# Autodesk Inventor assembly: Turntable-ArmConnection
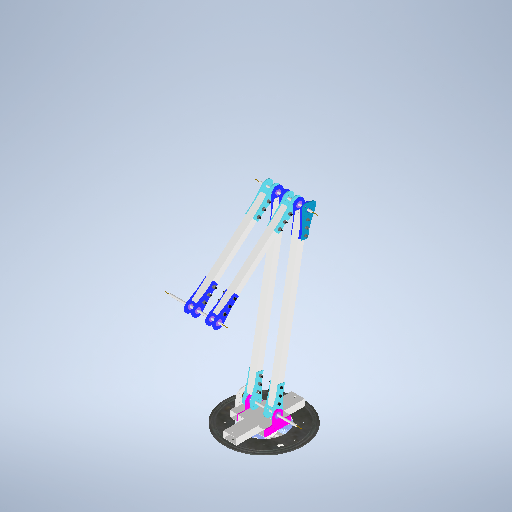
[picture p0: Inventor's stored thumbnail of the model, 512x512]
Saved by Autodesk Inventor 2025.1 (Build 291241000, 241)
## iProperties
Created: 2024-01-10
Part Number: Turntable-ArmConnection
Document SubType Name: Assembly
Designer: megan
Author: megan
## Documents named in this file (18)
- C:\Users\ejned\OneDrive - The Pennsylvania State University\BehrendURCMechanical\CAD\Apparatus\Arm Base\Arm.iam
- C:\Users\ejned\OneDrive - The Pennsylvania State University\BehrendURCMechanical\CAD\Apparatus\Arm Base\1544T3_Lubricated Turntable.ipt
- C:\Users\ejned\OneDrive - The Pennsylvania State University\BehrendURCMechanical\CAD\Apparatus\Arm Base\2inTubeBase.ipt
- C:\Users\ejned\OneDrive - The Pennsylvania State University\BehrendURCMechanical\CAD\Apparatus\Arm Base\1inTubeBase.ipt
- C:\Users\ejned\OneDrive - The Pennsylvania State University\BehrendURCMechanical\CAD\Apparatus\Arm Base\ArmPlateBase.ipt
- C:\Users\ejned\OneDrive - The Pennsylvania State University\BehrendURCMechanical\CAD\Apparatus\Arm Base\JointShaft.ipt
- C:\Users\ejned\OneDrive - The Pennsylvania State University\BehrendURCMechanical\CAD\Chassis V3\Arm Plate2.ipt
- C:\Users\ejned\OneDrive - The Pennsylvania State University\BehrendURCMechanical\CAD\Chassis V3\24in long 1in square tube.ipt
- C:\Users\ejned\OneDrive - The Pennsylvania State University\BehrendURCMechanical\CAD\Apparatus\Arm Base\8mmBearing.ipt
- C:\Users\ejned\OneDrive - The Pennsylvania State University\BehrendURCMechanical\CAD\Chassis V3\Arm Plate.ipt
- C:\Users\ejned\OneDrive - The Pennsylvania State University\BehrendURCMechanical\CAD\Chassis V3\14in long 1in square tube.ipt
- C:\Users\ejned\OneDrive - The Pennsylvania State University\BehrendURCMechanical\CAD\Chassis V3\Bolt Nut Washer assem.iam
- C:\Users\ejned\OneDrive - The Pennsylvania State University\BehrendURCMechanical\CAD\Apparatus\Arm Base\AP-0-02-baseAllTry2.iam
- C:\Users\ejned\OneDrive - The Pennsylvania State University\BehrendURCMechanical\CAD\Chassis V3\90107A011_316 Stainless Steel Washer.ipt
- C:\Users\ejned\OneDrive - The Pennsylvania State University\BehrendURCMechanical\CAD\Chassis V3\Arm Plate4.ipt
- C:\Users\ejned\OneDrive - The Pennsylvania State University\BehrendURCMechanical\CAD\Apparatus\91290A198_Alloy Steel Socket Head Screw.ipt
- C:\Users\ejned\OneDrive - The Pennsylvania State University\BehrendURCMechanical\CAD\Chassis V3\91831A011_18-8 Stainless Steel Nylon-Insert Locknut.ipt
- C:\Users\ejned\OneDrive - The Pennsylvania State University\BehrendURCMechanical\CAD\Apparatus\Arm Base\ArmPlateBase V2.ipt
## Components (76 placed, 15 different names)
1. 1544T3_Lubricated Turntable:1 — Mate:3, Mate:197, Mate:198, Mate:199, Mate:201
2. AP-0-02-baseAllTry2:1 [sub-assembly] — Mate:199
3. ArmPlateBase V2:1 — Rotational:1
4. ArmPlateBase:1 — Mate:57, Mate:58, Mate:59, Mate:60, Mate:63, Mate:65, Mate:271, Mate:272, Mate:273
5. ArmPlateBase:2 — Mate:61, Mate:62, Flush:5, Mate:66
6. arm plate:1 — Mate:22, Mate:73, Mate:74, Mate:142, Mate:143, Mate:150, Mate:151, Mate:152, Mate:153
7. arm plate:3 — Mate:80, Mate:81, Mate:204, Mate:207, Mate:236, Mate:237
8. arm plate:4 — Mate:49, Mate:50, Mate:51, Mate:213, Mate:262, Mate:264, Mate:266
9. arm plate:5 — Mate:67, Mate:68, Mate:69, Mate:77, Mate:78, Mate:154, Mate:155, Mate:156, Mate:157, Mate:168, Mate:169, Mate:284
10. arm plate:6 — Mate:70, Mate:71, Mate:72, Mate:79, Mate:82, Mate:283
11. arm plate:7 — Mate:84, Mate:86
12. arm plate:8 — Mate:83, Mate:85
13. arm plate:10 — Mate:93, Mate:104, Mate:105, Mate:170, Mate:171, Mate:172, Mate:173, Mate:174, Mate:175, Mate:283
14. arm plate:11 — Mate:95, Mate:101, Flush:7, Mate:159, Mate:284
15. arm plate:12 — Mate:97, Mate:103, Mate:160
16. arm plate:13 — Mate:106, Mate:107, Mate:111, Mate:115, Mate:117, Mate:124, Mate:188, Mate:189, Mate:190, Mate:191, Mate:192, Mate:193
17. arm plate:14 — Mate:108, Mate:109, Mate:114, Mate:122
18. arm plate:15 — Mate:110, Mate:111, Mate:116, Mate:120
19. arm plate:16 — Mate:112, Mate:113, Flush:9, Mate:118, Mate:182, Mate:183, Mate:184, Mate:185, Mate:186, Mate:187
20. arm plate:18 — Mate:226, Mate:227, Mate:228, Mate:229, Mate:230, Mate:231, Mate:232, Mate:233, Mate:234
21. arm plate:19 — Mate:235, Mate:236, Mate:237, Mate:243, Mate:244, Mate:245, Mate:247, Mate:248, Mate:251, Mate:252, Mate:253, Mate:255, Mate:256, Mate:258, Mate:260, Flush:13
22. arm plate:20 — Mate:268, Mate:269, Mate:270, Mate:275, Mate:276, Mate:277, Mate:278, Mate:279, Mate:280, Mate:281
23. 2inTubeBase:1 — Mate:3, Mate:4, Mate:54, Mate:55, Mate:56, Flush:3, Flush:4, Flush:5, Mate:197, Mate:198
24. 1inTubeBase:1 — Mate:54, Mate:55, Mate:61, Mate:62, Flush:4
25. 1inTubeBase:2 — Mate:4, Mate:56, Flush:3, Mate:57, Mate:58, Mate:59, Mate:60
26. 24in long 1in square tube:1 — Flush:2, Mate:67, Mate:68, Mate:69, Mate:70, Mate:71, Mate:72, Mate:86, Mate:200, Mate:268, Mate:274, Mate:275
27. 24in long 1in square tube:2 — Flush:2, Mate:49, Mate:50, Mate:51, Mate:73, Mate:74, Mate:85, Mate:204, Mate:207, Mate:274
28. 14in long 1in square tube:1 — Mate:101, Flush:7, Flush:8, Mate:106, Mate:107, Mate:110, Mate:115, Mate:116, Mate:159, Mate:227, Mate:228
29. 14in long 1in square tube:2 — Flush:8, Mate:103, Mate:104, Mate:105, Mate:108, Mate:109, Mate:112, Mate:113, Flush:9, Mate:114, Mate:160
30. 1inTubeBase:3 — Mate:271, Mate:272, Mate:273, Rotational:1
31. 91831A011_18-8 Stainless Steel Nylon-Insert Locknut:9 — Mate:264, Mate:265
32. 91831A011_18-8 Stainless Steel Nylon-Insert Locknut:8 — Mate:266, Mate:267
33. 91831A011_18-8 Stainless Steel Nylon-Insert Locknut:7 — Mate:258, Mate:259
34. 91831A011_18-8 Stainless Steel Nylon-Insert Locknut:6 — Mate:260, Mate:261
35. 91831A011_18-8 Stainless Steel Nylon-Insert Locknut:5 — Mate:262, Mate:263
36. 91831A011_18-8 Stainless Steel Nylon-Insert Locknut:4 — Mate:256, Mate:257
37. 90107A011_316 Stainless Steel Washer:4 — Mate:252, Mate:253, Mate:254
38. 91290A198_Alloy Steel Socket Head Screw:3 — Mate:250, Mate:251, Mate:259, Mate:265
39. 91290A198_Alloy Steel Socket Head Screw:2 — Mate:254, Mate:255, Mate:261, Mate:267
40. 91290A198_Alloy Steel Socket Head Screw:1 — Mate:248, Mate:249, Mate:257, Mate:263
41. 90107A011_316 Stainless Steel Washer:3 — Mate:243, Mate:244, Mate:245, Mate:246, Mate:249
42. 90107A011_316 Stainless Steel Washer:2 — Mate:246, Mate:247, Mate:250
43. Bolt Nut Washer assem:24 [sub-assembly] — Mate:192, Mate:193
44. Bolt Nut Washer assem:21 [sub-assembly] — Mate:184, Mate:185
45. Bolt Nut Washer assem:20 [sub-assembly] — Mate:188, Mate:189
46. Bolt Nut Washer assem:19 [sub-assembly] — Mate:182, Mate:183
47. Bolt Nut Washer assem:18 [sub-assembly] — Mate:190, Mate:191
48. Bolt Nut Washer assem:17 [sub-assembly] — Mate:186, Mate:187
49. Bolt Nut Washer assem:16 [sub-assembly] — Mate:231, Mate:234
50. Bolt Nut Washer assem:15 [sub-assembly] — Mate:229, Mate:230
51. Bolt Nut Washer assem:14 [sub-assembly] — Mate:170, Mate:171
52. Bolt Nut Washer assem:13 [sub-assembly] — Mate:172, Mate:173
53. Bolt Nut Washer assem:11 [sub-assembly] — Mate:174, Mate:175
54. Bolt Nut Washer assem:10 [sub-assembly] — Mate:168, Mate:169
55. Bolt Nut Washer assem:9 [sub-assembly] — Mate:232, Mate:233
56. Bolt Nut Washer assem:8 [sub-assembly] — Mate:155, Mate:156
57. Bolt Nut Washer assem:7 [sub-assembly] — Mate:154, Mate:157
58. Bolt Nut Washer assem:6 [sub-assembly] — Mate:152, Mate:153
59. Bolt Nut Washer assem:5 [sub-assembly] — Mate:150, Mate:151
60. Bolt Nut Washer assem:4 [sub-assembly] — Mate:276, Mate:278
61. Bolt Nut Washer assem:3 [sub-assembly] — Mate:270, Mate:279, Mate:281
62. Bolt Nut Washer assem:2 [sub-assembly] — Mate:277, Mate:280
63. Bolt Nut Washer assem:1 [sub-assembly] — Mate:142, Mate:143
64. 8mmBearing:1 — Mate:36, Mate:66
65. 8mmBearing:2 — Mate:37, Mate:65
66. 8mmBearing:4 — Mate:77, Mate:78, Mate:87
67. 8mmBearing:5 — Mate:79, Mate:82
68. 8mmBearing:6 — Mate:80, Mate:81, Mate:203, Mate:235
69. 8mmBearing:7 — Mate:124, Mate:125
70. 8mmBearing:8 — Mate:120, Mate:121
71. 8mmBearing:9 — Mate:118, Mate:119, Flush:12
72. 8mmBearing:10 — Mate:122, Mate:123
73. 8mmBearing:11 — Mate:212, Mate:213
74. JointShaft:1 — Mate:22, Mate:36, Mate:37, Mate:63, Mate:83, Mate:84, Mate:269
75. JointShaft:2 — Mate:87, Mate:93, Mate:95, Mate:97, Mate:203, Mate:212, Mate:226, Flush:13
76. JointShaft:3 — Mate:117, Mate:119, Mate:121, Mate:123, Mate:125, Flush:12
## Relationships (171: Mate 161, Flush 9, RevoluteJoint 1)
- Mate:3: 1544T3_Lubricated Turntable:1 ↔ 2inTubeBase:1
- Mate:4: 2inTubeBase:1 ↔ 1inTubeBase:2
- Mate:22: arm plate:1 ↔ JointShaft:1
- Mate:36: 8mmBearing:1 ↔ JointShaft:1
- Mate:37: 8mmBearing:2 ↔ JointShaft:1
- Flush:2: 24in long 1in square tube:1 ↔ 24in long 1in square tube:2
- Mate:49: arm plate:4 ↔ 24in long 1in square tube:2
- Mate:50: arm plate:4 ↔ 24in long 1in square tube:2
- Mate:51: arm plate:4 ↔ 24in long 1in square tube:2
- Mate:54: 2inTubeBase:1 ↔ 1inTubeBase:1
- Mate:55: 2inTubeBase:1 ↔ 1inTubeBase:1
- Mate:56: 2inTubeBase:1 ↔ 1inTubeBase:2
- Flush:3: 2inTubeBase:1 ↔ 1inTubeBase:2
- Mate:57: ArmPlateBase:1 ↔ 1inTubeBase:2
- Mate:58: ArmPlateBase:1 ↔ 1inTubeBase:2
- Mate:59: ArmPlateBase:1 ↔ 1inTubeBase:2
- Mate:60: ArmPlateBase:1 ↔ 1inTubeBase:2
- Mate:61: ArmPlateBase:2 ↔ 1inTubeBase:1
- Mate:62: ArmPlateBase:2 ↔ 1inTubeBase:1
- Flush:4: 2inTubeBase:1 ↔ 1inTubeBase:1
- Flush:5: ArmPlateBase:2 ↔ 2inTubeBase:1
- Mate:63: ArmPlateBase:1 ↔ JointShaft:1
- Mate:65: ArmPlateBase:1 ↔ 8mmBearing:2
- Mate:66: ArmPlateBase:2 ↔ 8mmBearing:1
- Mate:67: arm plate:5 ↔ 24in long 1in square tube:1
- Mate:68: arm plate:5 ↔ 24in long 1in square tube:1
- Mate:69: arm plate:5 ↔ 24in long 1in square tube:1
- Mate:70: arm plate:6 ↔ 24in long 1in square tube:1
- Mate:71: arm plate:6 ↔ 24in long 1in square tube:1
- Mate:72: arm plate:6 ↔ 24in long 1in square tube:1
- Mate:73: arm plate:1 ↔ 24in long 1in square tube:2
- Mate:74: arm plate:1 ↔ 24in long 1in square tube:2
- Mate:77: arm plate:5 ↔ 8mmBearing:4
- Mate:78: arm plate:5 ↔ 8mmBearing:4
- Mate:79: arm plate:6 ↔ 8mmBearing:5
- Mate:80: arm plate:3 ↔ 8mmBearing:6
- Mate:81: arm plate:3 ↔ 8mmBearing:6
- Mate:82: arm plate:6 ↔ 8mmBearing:5
- Mate:83: arm plate:8 ↔ JointShaft:1
- Mate:84: arm plate:7 ↔ JointShaft:1
- Mate:85: arm plate:8 ↔ 24in long 1in square tube:2
- Mate:86: arm plate:7 ↔ 24in long 1in square tube:1
- Mate:87: 8mmBearing:4 ↔ JointShaft:2
- Mate:93: arm plate:10 ↔ JointShaft:2
- Mate:95: arm plate:11 ↔ JointShaft:2
- Mate:97: arm plate:12 ↔ JointShaft:2
- Mate:101: arm plate:11 ↔ 14in long 1in square tube:1
- Flush:7: arm plate:11 ↔ 14in long 1in square tube:1
- Flush:8: 14in long 1in square tube:1 ↔ 14in long 1in square tube:2
- Mate:103: arm plate:12 ↔ 14in long 1in square tube:2
- Mate:104: arm plate:10 ↔ 14in long 1in square tube:2
- Mate:105: arm plate:10 ↔ 14in long 1in square tube:2
- Mate:106: arm plate:13 ↔ 14in long 1in square tube:1
- Mate:107: arm plate:13 ↔ 14in long 1in square tube:1
- Mate:108: arm plate:14 ↔ 14in long 1in square tube:2
- Mate:109: arm plate:14 ↔ 14in long 1in square tube:2
- Mate:110: arm plate:15 ↔ 14in long 1in square tube:1
- Mate:111: arm plate:13 ↔ arm plate:15
- Mate:112: arm plate:16 ↔ 14in long 1in square tube:2
- Mate:113: arm plate:16 ↔ 14in long 1in square tube:2
- Flush:9 (-2 mm): arm plate:16 ↔ 14in long 1in square tube:2
- Mate:114: arm plate:14 ↔ 14in long 1in square tube:2
- Mate:115: arm plate:13 ↔ 14in long 1in square tube:1
- Mate:116: arm plate:15 ↔ 14in long 1in square tube:1
- Mate:117: arm plate:13 ↔ JointShaft:3
- Mate:118: arm plate:16 ↔ 8mmBearing:9
- Mate:119: 8mmBearing:9 ↔ JointShaft:3
- Mate:120: arm plate:15 ↔ 8mmBearing:8
- Mate:121: 8mmBearing:8 ↔ JointShaft:3
- Mate:122: arm plate:14 ↔ 8mmBearing:10
- Mate:123: 8mmBearing:10 ↔ JointShaft:3
- Mate:124: arm plate:13 ↔ 8mmBearing:7
- Mate:125: 8mmBearing:7 ↔ JointShaft:3
- Mate:142: arm plate:1 ↔ Bolt Nut Washer assem:1
- Mate:143: arm plate:1 ↔ Bolt Nut Washer assem:1
- Mate:150: arm plate:1 ↔ Bolt Nut Washer assem:5
- Mate:151: arm plate:1 ↔ Bolt Nut Washer assem:5
- Mate:152: arm plate:1 ↔ Bolt Nut Washer assem:6
- Mate:153: arm plate:1 ↔ Bolt Nut Washer assem:6
- Mate:154: arm plate:5 ↔ Bolt Nut Washer assem:7
- Mate:155: arm plate:5 ↔ Bolt Nut Washer assem:8
- Mate:156: arm plate:5 ↔ Bolt Nut Washer assem:8
- Mate:157: arm plate:5 ↔ Bolt Nut Washer assem:7
- Mate:159: arm plate:11 ↔ 14in long 1in square tube:1
- Mate:160: arm plate:12 ↔ 14in long 1in square tube:2
- Mate:168: arm plate:5 ↔ Bolt Nut Washer assem:10
- Mate:169: arm plate:5 ↔ Bolt Nut Washer assem:10
- Mate:170: arm plate:10 ↔ Bolt Nut Washer assem:14
- Mate:171: arm plate:10 ↔ Bolt Nut Washer assem:14
- Mate:172: arm plate:10 ↔ Bolt Nut Washer assem:13
- Mate:173: arm plate:10 ↔ Bolt Nut Washer assem:13
- Mate:174: arm plate:10 ↔ Bolt Nut Washer assem:11
- Mate:175: arm plate:10 ↔ Bolt Nut Washer assem:11
- Mate:182: arm plate:16 ↔ Bolt Nut Washer assem:19
- Mate:183: arm plate:16 ↔ Bolt Nut Washer assem:19
- Mate:184: arm plate:16 ↔ Bolt Nut Washer assem:21
- Mate:185: arm plate:16 ↔ Bolt Nut Washer assem:21
- Mate:186: arm plate:16 ↔ Bolt Nut Washer assem:17
- Mate:187: arm plate:16 ↔ Bolt Nut Washer assem:17
- Mate:188: arm plate:13 ↔ Bolt Nut Washer assem:20
- Mate:189: arm plate:13 ↔ Bolt Nut Washer assem:20
- Mate:190: arm plate:13 ↔ Bolt Nut Washer assem:18
- Mate:191: arm plate:13 ↔ Bolt Nut Washer assem:18
- Mate:192: arm plate:13 ↔ Bolt Nut Washer assem:24
- Mate:193: arm plate:13 ↔ Bolt Nut Washer assem:24
- Mate:197: 1544T3_Lubricated Turntable:1 ↔ 2inTubeBase:1
- Mate:198: 1544T3_Lubricated Turntable:1 ↔ 2inTubeBase:1
- Mate:199: 1544T3_Lubricated Turntable:1 ↔ AP-0-02-baseAllTry2:1
- Mate:200: 24in long 1in square tube:1
- Mate:201: 1544T3_Lubricated Turntable:1
- Mate:203: 8mmBearing:6 ↔ JointShaft:2
- Mate:204: arm plate:3 ↔ 24in long 1in square tube:2
- Mate:207: arm plate:3 ↔ 24in long 1in square tube:2
- Mate:212: 8mmBearing:11 ↔ JointShaft:2
- Mate:213: arm plate:4 ↔ 8mmBearing:11
- Flush:12 (-12.7 mm): 8mmBearing:9 ↔ JointShaft:3
- Mate:226: arm plate:18 ↔ JointShaft:2
- Mate:227: arm plate:18 ↔ 14in long 1in square tube:1
- Mate:228: arm plate:18 ↔ 14in long 1in square tube:1
- Mate:229: arm plate:18 ↔ Bolt Nut Washer assem:15
- Mate:230: arm plate:18 ↔ Bolt Nut Washer assem:15
- Mate:231: arm plate:18 ↔ Bolt Nut Washer assem:16
- Mate:232: arm plate:18 ↔ Bolt Nut Washer assem:9
- Mate:233: arm plate:18 ↔ Bolt Nut Washer assem:9
- Mate:234: arm plate:18 ↔ Bolt Nut Washer assem:16
- Mate:235: arm plate:19 ↔ 8mmBearing:6
- Mate:236 (6.35 mm): arm plate:3 ↔ arm plate:19
- Mate:237: arm plate:3 ↔ arm plate:19
- Mate:243: arm plate:19 ↔ 90107A011_316 Stainless Steel Washer:3
- Mate:244: arm plate:19 ↔ 90107A011_316 Stainless Steel Washer:3
- Mate:245: arm plate:19 ↔ 90107A011_316 Stainless Steel Washer:3
- Mate:246: 90107A011_316 Stainless Steel Washer:3 ↔ 90107A011_316 Stainless Steel Washer:2
- Mate:247: arm plate:19 ↔ 90107A011_316 Stainless Steel Washer:2
- Mate:248: arm plate:19 ↔ 91290A198_Alloy Steel Socket Head Screw:1
- Mate:249: 91290A198_Alloy Steel Socket Head Screw:1 ↔ 90107A011_316 Stainless Steel Washer:3
- Mate:250: 91290A198_Alloy Steel Socket Head Screw:3 ↔ 90107A011_316 Stainless Steel Washer:2
- Mate:251: arm plate:19 ↔ 91290A198_Alloy Steel Socket Head Screw:3
- Mate:252: arm plate:19 ↔ 90107A011_316 Stainless Steel Washer:4
- Mate:253: arm plate:19 ↔ 90107A011_316 Stainless Steel Washer:4
- Mate:254: 90107A011_316 Stainless Steel Washer:4 ↔ 91290A198_Alloy Steel Socket Head Screw:2
- Mate:255: arm plate:19 ↔ 91290A198_Alloy Steel Socket Head Screw:2
- Mate:256: arm plate:19 ↔ 91831A011_18-8 Stainless Steel Nylon-Insert Locknut:4
- Mate:257: 91831A011_18-8 Stainless Steel Nylon-Insert Locknut:4 ↔ 91290A198_Alloy Steel Socket Head Screw:1
- Mate:258: arm plate:19 ↔ 91831A011_18-8 Stainless Steel Nylon-Insert Locknut:7
- Mate:259: 91831A011_18-8 Stainless Steel Nylon-Insert Locknut:7 ↔ 91290A198_Alloy Steel Socket Head Screw:3
- Mate:260: arm plate:19 ↔ 91831A011_18-8 Stainless Steel Nylon-Insert Locknut:6
- Mate:261: 91831A011_18-8 Stainless Steel Nylon-Insert Locknut:6 ↔ 91290A198_Alloy Steel Socket Head Screw:2
- Mate:262: arm plate:4 ↔ 91831A011_18-8 Stainless Steel Nylon-Insert Locknut:5
- Mate:263: 91831A011_18-8 Stainless Steel Nylon-Insert Locknut:5 ↔ 91290A198_Alloy Steel Socket Head Screw:1
- Mate:264: arm plate:4 ↔ 91831A011_18-8 Stainless Steel Nylon-Insert Locknut:9
- Mate:265: 91831A011_18-8 Stainless Steel Nylon-Insert Locknut:9 ↔ 91290A198_Alloy Steel Socket Head Screw:3
- Mate:266: arm plate:4 ↔ 91831A011_18-8 Stainless Steel Nylon-Insert Locknut:8
- Mate:267: 91831A011_18-8 Stainless Steel Nylon-Insert Locknut:8 ↔ 91290A198_Alloy Steel Socket Head Screw:2
- Mate:268: arm plate:20 ↔ 24in long 1in square tube:1
- Mate:269: arm plate:20 ↔ JointShaft:1
- Mate:270: arm plate:20 ↔ Bolt Nut Washer assem:3
- Mate:271: ArmPlateBase:1 ↔ 1inTubeBase:3
- Mate:272: ArmPlateBase:1 ↔ 1inTubeBase:3
- Mate:273: ArmPlateBase:1 ↔ 1inTubeBase:3
- Mate:274 (57.15 mm): 24in long 1in square tube:1 ↔ 24in long 1in square tube:2
- Mate:275: arm plate:20 ↔ 24in long 1in square tube:1
- Mate:276: arm plate:20 ↔ Bolt Nut Washer assem:4
- Mate:277: arm plate:20 ↔ Bolt Nut Washer assem:2
- Mate:278: arm plate:20 ↔ Bolt Nut Washer assem:4
- Mate:279: arm plate:20 ↔ Bolt Nut Washer assem:3
- Mate:280: arm plate:20 ↔ Bolt Nut Washer assem:2
- Mate:281: arm plate:20 ↔ Bolt Nut Washer assem:3
- Flush:13 (12.7 mm): arm plate:19 ↔ JointShaft:2
- Mate:283 (9.398 mm): arm plate:6 ↔ arm plate:10
- Mate:284 (9.398 mm): arm plate:5 ↔ arm plate:11
- Rotational:1 [RevoluteJoint]: ArmPlateBase V2:1 ↔ 1inTubeBase:3
